# Autodesk Inventor assembly: Robot_Part_Braccio Robotic Arm
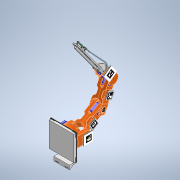
[picture p0: Inventor's stored thumbnail of the model, 180x180]
Saved by Autodesk Inventor 2022.2 (Build 262287010, 287A)
## iProperties
Created: 2023-04-03
Part Number: Robot_Part_Braccio Robotic Arm
Document SubType Name: Assembly
Designer: ppovolni
Sending System: SolidWorks 2018
Last Author: 86136
Last Saved: 2023-04-21
UNIT_OF_MEASURE: - 无 -
总图号: MT000-01
名称: 组件(迈通)
数量: 0
Author: ppovolni
## Documents named in this file (28)
- D:\3_Local_Projekte\ALF\alf_nmr_magnetometer\2_Project_Motiontracking_Robotarm\CAD\Baugruppe_Braccio\Robot_Part_Braccio Robotic Arm.iam
- D:\3_Local_Projekte\ALF\alf_nmr_magnetometer\2_Project_Motiontracking_Robotarm\CAD\Baugruppe_Braccio\1_Robot_Mechanics\Robot_Part_BASE-INFERIORE_33 (2).ipt
- D:\3_Local_Projekte\ALF\alf_nmr_magnetometer\2_Project_Motiontracking_Robotarm\CAD\Baugruppe_Braccio\1_Robot_Mechanics\Robot_Part_COPERCHIO-BASE-NEW_1 (2).ipt
- D:\3_Local_Projekte\ALF\alf_nmr_magnetometer\2_Project_Motiontracking_Robotarm\CAD\Baugruppe_Braccio\1_Robot_Mechanics\Robot_Part_ASTA-BRACCIO-PROVA_1 (2).ipt
- D:\3_Local_Projekte\ALF\alf_nmr_magnetometer\2_Project_Motiontracking_Robotarm\CAD\Baugruppe_Braccio\1_Robot_Mechanics\Robot_Part_DITO2_1dzdfd (2).ipt
- D:\3_Local_Projekte\ALF\alf_nmr_magnetometer\2_Project_Motiontracking_Robotarm\CAD\Baugruppe_Braccio\1_Robot_Mechanics\Robot_Part_GUIDA-MOTORE-MANO_1 (2).ipt
- D:\3_Local_Projekte\ALF\alf_nmr_magnetometer\2_Project_Motiontracking_Robotarm\CAD\Baugruppe_Braccio\1_Robot_Mechanics\Robot_Part_INGRANAGGIO-BRACCIO-22_1 (2).ipt
- D:\3_Local_Projekte\ALF\alf_nmr_magnetometer\2_Project_Motiontracking_Robotarm\CAD\Baugruppe_Braccio\1_Robot_Mechanics\Robot_Part_SERVO (1).ipt
- D:\3_Local_Projekte\ALF\alf_nmr_magnetometer\2_Project_Motiontracking_Robotarm\CAD\Baugruppe_Braccio\1_Robot_Mechanics\Robot_Part_STAFFA-POLSO_36 (2).ipt
- D:\3_Local_Projekte\ALF\alf_nmr_magnetometer\2_Project_Motiontracking_Robotarm\CAD\Baugruppe_Braccio\1_Robot_Mechanics\Robot_Part_SUPP. BASE Ver 01 (1).ipt
- D:\3_Local_Projekte\ALF\alf_nmr_magnetometer\2_Project_Motiontracking_Robotarm\CAD\Baugruppe_Braccio\1_Robot_Mechanics\Robot_Part_SUPP. MOTORE BASE Ver01 (2).ipt
- D:\3_Local_Projekte\ALF\alf_nmr_magnetometer\2_Project_Motiontracking_Robotarm\CAD\Baugruppe_Braccio\1_Robot_Mechanics\Robot_Part_SUPP-MANO (1).ipt
- D:\3_Local_Projekte\ALF\alf_nmr_magnetometer\2_Project_Motiontracking_Robotarm\CAD\Baugruppe_Braccio\1_Robot_Mechanics\Robot_Part_TIRANTI_1 (2).ipt
- D:\3_Local_Projekte\ALF\alf_nmr_magnetometer\2_Project_Motiontracking_Robotarm\CAD\Baugruppe_Braccio\1_Robot_Mechanics\Robot_Part_SR311外观.iam
- D:\3_Local_Projekte\ALF\alf_nmr_magnetometer\2_Project_Motiontracking_Robotarm\CAD\Baugruppe_Braccio\1_Robot_Mechanics\Robot_Part_SR431外观.iam
- D:\3_Local_Projekte\ALF\alf_nmr_magnetometer\2_Project_Motiontracking_Robotarm\CAD\Baugruppe_Braccio\1_Robot_Mechanics\Robot_Part_INGRANAGGIO-BRACCIO-22_1 (1).ipt
- D:\3_Local_Projekte\ALF\alf_nmr_magnetometer\2_Project_Motiontracking_Robotarm\CAD\Baugruppe_Braccio\1_Robot_Mechanics\Robot_Part_Bauteil150.ipt
- D:\3_Local_Projekte\ALF\alf_nmr_magnetometer\2_Project_Motiontracking_Robotarm\CAD\Baugruppe_Braccio\3_Hallsensor_Holder\Assembly_Adapter_Wrist_220mm.iam
- D:\3_Local_Projekte\ALF\alf_nmr_magnetometer\2_Project_Motiontracking_Robotarm\CAD\Potentiometer\Baugruppe_Poti.iam
- D:\3_Local_Projekte\ALF\alf_nmr_magnetometer\2_Project_Motiontracking_Robotarm\CAD\Potentiometer\Halterung_Robot.ipt
- D:\3_Local_Projekte\ALF\alf_nmr_magnetometer\2_Project_Motiontracking_Robotarm\CAD\Baugruppe_Braccio\4_ownParts\Adapter_Plate_12mm.ipt
- D:\3_Local_Projekte\ALF\alf_nmr_magnetometer\2_Project_Motiontracking_Robotarm\CAD\Baugruppe_Braccio\4_ownParts\Positioning_Robot.ipt
- D:\3_Local_Projekte\ALF\alf_nmr_magnetometer\2_Project_Motiontracking_Robotarm\CAD\Baugruppe_Braccio\2_Aruco_Marker\Aruco_Wrist_final_id3.ipt
- D:\3_Local_Projekte\ALF\alf_nmr_magnetometer\2_Project_Motiontracking_Robotarm\CAD\Baugruppe_Braccio\2_Aruco_Marker\Aruco_Shoulder_final_id2.ipt
- D:\3_Local_Projekte\ALF\alf_nmr_magnetometer\2_Project_Motiontracking_Robotarm\CAD\Baugruppe_Braccio\2_Aruco_Marker\Aruco_Shoulder_final_id1.ipt
- D:\3_Local_Projekte\ALF\alf_nmr_magnetometer\2_Project_Motiontracking_Robotarm\CAD\Baugruppe_Braccio\2_Aruco_Marker\Aruco_Basis_final_id0.ipt
- D:\3_Local_Projekte\ALF\alf_nmr_magnetometer\2_Project_Motiontracking_Robotarm\CAD\Baugruppe_Braccio\4_ownParts\Kabel_braccio.ipt
- D:\3_Local_Projekte\ALF\alf_nmr_magnetometer\2_Project_Motiontracking_Robotarm\CAD\Baugruppe_Braccio\4_ownParts\Cover_Robot_Motor_Shoulder.ipt
## Components (42 placed, 27 different names)
1. Baugruppe_Poti:1 [sub-assembly] — Fluchtend:1, Fluchtend:2, Passend:13, Passend:15
2. Halterung_Robot:1 — Passend:14, Passend:15
3. Adapter_Plate_12mm:1 — Passend:18, Passend:19, Passend:20
4. Positioning_Robot:1 — Passend:16, Passend:17, Winkel:9, Passend:18, Passend:19, Passend:20
5. Kabel_braccio:1 — Fluchtend:3, Passend:21
6. Cover_Robot_Motor_Shoulder:1 — Fluchtend:4, Fluchtend:5
7. BASE-INFERIORE_33 (2):1 — Passend:4, Fluchtend:1, Passend:13, Passend:16, Passend:17
8. COPERCHIO-BASE-NEW_1 (2):1 — Passend:14
9. ASTA-BRACCIO-PROVA_1 (2):1 — Passend:11, Winkel:7
10. SERVO (1):1
11. STAFFA-POLSO_36 (2):1 — Passend:5, Winkel:1, Passend:8, Passend:9
12. SUPP. BASE Ver 01 (1):1 — Tangential:1
13. SUPP. MOTORE BASE Ver01 (2):1
14. ASTA-BRACCIO-PROVA_1 (2):2
15. SR311外观:1 [sub-assembly] — Passend:6
16. SR431外观:1 [sub-assembly]
17. SR431外观:2 [sub-assembly]
18. SR431外观:3 [sub-assembly] — Passend:2
19. ASTA-BRACCIO-PROVA_1 (2):4 — Passend:21
20. ASTA-BRACCIO-PROVA_1 (2):5 — Passend:10, Winkel:6, Fluchtend:4, Fluchtend:5
21. SERVO (1):3 — Passend:3
22. SERVO (1):4
23. SR431外观:4 [sub-assembly] — Passend:1
24. SERVO (1):5
25. Robot_Part_Bauteil150
26. DITO2_1dzdfd (2):1
27. GUIDA-MOTORE-MANO_1 (2):1
28. INGRANAGGIO-BRACCIO-22_1 (2):1
29. SUPP-MANO (1):1
30. TIRANTI_1 (2):1
31. SR311外观:2 [sub-assembly]
32. GUIDA-MOTORE-MANO_1 (2):2
33. TIRANTI_1 (2):2
34. INGRANAGGIO-BRACCIO-22_1 (1):1
35. TIRANTI_1 (2):3
36. DITO2_1dzdfd (2):2
37. TIRANTI_1 (2):4
38. Aruco_Shoulder_final_id1:1 — Passend:11, Winkel:7, Passend:12
39. Aruco_Basis_final_id0:1 — Winkel:2, Passend:7, Winkel:5, Tangential:1, Winkel:9
40. Aruco_Shoulder_final_id2:1 — Passend:10, Winkel:6
41. Aruco_Wrist_final_id3:1 — Passend:8, Passend:9
42. Assembly_Adapter_Wrist_220mm:1 [sub-assembly] — Passend:5, Passend:6, Winkel:1, Fluchtend:3
## Relationships (34: Mate 21, Angle 7, Flush 5, Tangent 1)
- Passend:1 [Mate]: SR431外观:4
- Passend:2 [Mate]: SR431外观:3
- Passend:3 [Mate]: SERVO (1):3
- Passend:4 [Mate]: BASE-INFERIORE_33 (2):1
- Passend:5 [Mate]: STAFFA-POLSO_36 (2):1 ↔ Assembly_Adapter_Wrist_220mm:1
- Passend:6 [Mate]: SR311外观:1 ↔ Assembly_Adapter_Wrist_220mm:1
- Winkel:1 [Angle] (180 deg): STAFFA-POLSO_36 (2):1 ↔ Assembly_Adapter_Wrist_220mm:1
- Winkel:2 [Angle] (0 deg): Aruco_Basis_final_id0:1
- Passend:7 [Mate]: Aruco_Basis_final_id0:1
- Winkel:5 [Angle] (0 deg): Aruco_Basis_final_id0:1
- Passend:8 [Mate]: STAFFA-POLSO_36 (2):1 ↔ Aruco_Wrist_final_id3:1
- Passend:9 [Mate]: STAFFA-POLSO_36 (2):1 ↔ Aruco_Wrist_final_id3:1
- Tangential:1: SUPP. BASE Ver 01 (1):1 ↔ Aruco_Basis_final_id0:1
- Passend:10 [Mate]: ASTA-BRACCIO-PROVA_1 (2):5 ↔ Aruco_Shoulder_final_id2:1
- Winkel:6 [Angle] (180 deg): ASTA-BRACCIO-PROVA_1 (2):5 ↔ Aruco_Shoulder_final_id2:1
- Passend:11 [Mate]: ASTA-BRACCIO-PROVA_1 (2):1 ↔ Aruco_Shoulder_final_id1:1
- Winkel:7 [Angle] (0 deg): ASTA-BRACCIO-PROVA_1 (2):1 ↔ Aruco_Shoulder_final_id1:1
- Passend:12 [Mate]: Aruco_Shoulder_final_id1:1
- Winkel:8 [Angle] (0 deg)
- Fluchtend:1 [Flush] (12 mm): Baugruppe_Poti:1 ↔ BASE-INFERIORE_33 (2):1
- Fluchtend:2 [Flush]: Baugruppe_Poti:1
- Passend:13 [Mate] (90 mm): Baugruppe_Poti:1 ↔ BASE-INFERIORE_33 (2):1
- Passend:14 [Mate]: Halterung_Robot:1 ↔ COPERCHIO-BASE-NEW_1 (2):1
- Passend:15 [Mate] (0.5 mm): Baugruppe_Poti:1 ↔ Halterung_Robot:1
- Passend:16 [Mate]: Positioning_Robot:1 ↔ BASE-INFERIORE_33 (2):1
- Passend:17 [Mate]: Positioning_Robot:1 ↔ BASE-INFERIORE_33 (2):1
- Winkel:9 [Angle] (0 deg): Positioning_Robot:1 ↔ Aruco_Basis_final_id0:1
- Passend:18 [Mate]: Adapter_Plate_12mm:1 ↔ Positioning_Robot:1
- Passend:19 [Mate]: Adapter_Plate_12mm:1 ↔ Positioning_Robot:1
- Passend:20 [Mate]: Adapter_Plate_12mm:1 ↔ Positioning_Robot:1
- Fluchtend:3 [Flush]: Kabel_braccio:1 ↔ Assembly_Adapter_Wrist_220mm:1
- Passend:21 [Mate]: Kabel_braccio:1 ↔ ASTA-BRACCIO-PROVA_1 (2):4
- Fluchtend:4 [Flush]: Cover_Robot_Motor_Shoulder:1 ↔ ASTA-BRACCIO-PROVA_1 (2):5
- Fluchtend:5 [Flush]: Cover_Robot_Motor_Shoulder:1 ↔ ASTA-BRACCIO-PROVA_1 (2):5
